# Autodesk Inventor assembly: Assembly
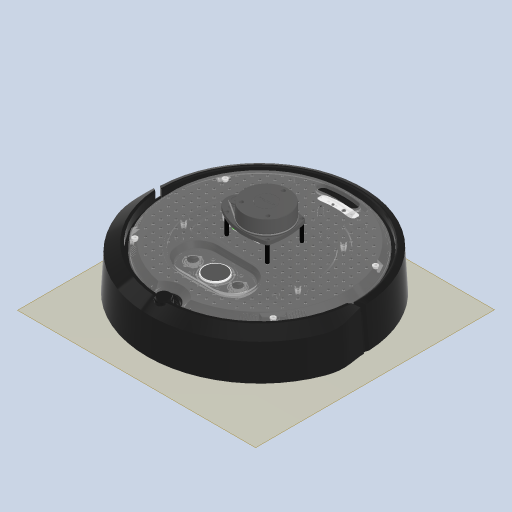
[picture p0: Inventor's stored thumbnail of the model, 512x512]
Saved by Autodesk Inventor 2024 (Build 280153000, 153)
## iProperties
Created: 2023-11-21
Part Number: Assembly
Document SubType Name: Assembly
Designer: Greg
Author: Greg
## Documents named in this file (3)
- C:\Users\Greg\Documents\Inventor\Capstone\Assembly.iam
- C:\Users\Greg\Documents\Inventor\Capstone\iRobot_Create_3_Public_Model\iRobot_Create_3_Public_Model.iam
- C:\Users\Greg\Documents\Inventor\Capstone\RPLIDAR A1M8\RPLIDAR A1M8.iam
## Components (2 placed, 2 different names)
1. iRobot_Create_3_Public_Model:1 [sub-assembly] — Angle:1, Tangent:1, Insert:1
2. RPLIDAR A1M8:1 [sub-assembly] — Insert:1
## Relationships (3: Angle 1, Tangent 1, Insert 1)
- Angle:1 (0 deg): iRobot_Create_3_Public_Model:1
- Tangent:1: iRobot_Create_3_Public_Model:1
- Insert:1: iRobot_Create_3_Public_Model:1 ↔ RPLIDAR A1M8:1
